# Autodesk Inventor assembly: RaspberryPi
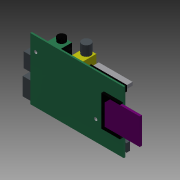
[picture p0: Inventor's stored thumbnail of the model, 180x180]
Saved by Autodesk Inventor 2014 (Build 180170000, 170)
## iProperties
Created: 2013-05-24
Part Number: RaspberryPi
Document SubType Name: Assembly
Designer: hartmann
Author: hartmann
## Documents named in this file (3)
- C:\Dokumente und Einstellungen\hartmann\Desktop\RaspberryPi\RaspberryPi.iam
- C:\Dokumente und Einstellungen\hartmann\Desktop\RaspberryPi\PCB.ipt
- C:\Dokumente und Einstellungen\hartmann\Desktop\RaspberryPi\SD.ipt
## Components (2 placed, 2 different names)
1. PCB:1 — Passend:1, Passend:2, Passend:3
2. SD:1 — Passend:1, Passend:2, Passend:3
## Relationships (3: Mate 3)
- Passend:1 [Mate]: PCB:1 ↔ SD:1
- Passend:2 [Mate]: PCB:1 ↔ SD:1
- Passend:3 [Mate]: PCB:1 ↔ SD:1
